# Autodesk Inventor assembly: Intake 1
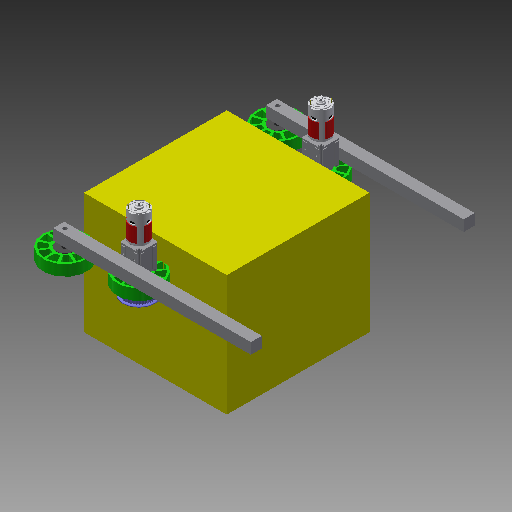
[picture p0: Inventor's stored thumbnail of the model, 512x512]
Saved by Autodesk Inventor 2018 (Build 220112000, 112)
## iProperties
Created: 2018-01-18
Part Number: Intake 1
Document SubType Name: Assembly
Designer: Apple
Author: Apple
## Documents named in this file (5)
- C:\Users\Apple\Documents\Inventor\2018 PowerUp\Cube Intake\Intake 1.iam
- C:\Users\Apple\Documents\Inventor\2018 PowerUp\2018 power cube.ipt
- C:\Users\Apple\Documents\Inventor\2018 PowerUp\Cube Intake\Sport57 with Redline and 4inc wheel.iam
- C:\Users\Apple\Documents\Inventor\2018 PowerUp\Cube Intake\Intake Arm.ipt
- C:\Users\Apple\Documents\Inventor\2018 PowerUp\AndyMark\am-3480+4IN+500Hex+Bore+Compliant+Wheel.ipt
## Components (7 placed, 4 different names)
1. 2018 power cube:1 — Mate:5, Mate:6, Flush:9
2. Sport57 with Redline and 4inc wheel:1 [sub-assembly] — Mate:1, Flush:2, Flush:3, Flush:4, Mate:6
3. Sport57 with Redline and 4inc wheel:2 [sub-assembly] — Mate:3, Flush:5, Flush:6, Mate:5, Mate:7
4. Intake Arm:1 — Mate:1, Flush:2, Flush:3, Mate:2, Flush:7, Flush:8
5. am-3480+4IN+500Hex+Bore+Compliant+Wheel:1 — Flush:4, Mate:2
6. Intake Arm:2 — Mate:3, Flush:5, Mate:4, Mate:7, Flush:7, Flush:8, Flush:9
7. am-3480+4IN+500Hex+Bore+Compliant+Wheel:2 — Mate:4, Flush:6
## Relationships (15: Flush 8, Mate 7)
- Mate:1: Sport57 with Redline and 4inc wheel:1 ↔ Intake Arm:1
- Flush:2: Sport57 with Redline and 4inc wheel:1 ↔ Intake Arm:1
- Flush:3 (127 mm): Sport57 with Redline and 4inc wheel:1 ↔ Intake Arm:1
- Flush:4: Sport57 with Redline and 4inc wheel:1 ↔ am-3480+4IN+500Hex+Bore+Compliant+Wheel:1
- Mate:2: Intake Arm:1 ↔ am-3480+4IN+500Hex+Bore+Compliant+Wheel:1
- Mate:3: Sport57 with Redline and 4inc wheel:2 ↔ Intake Arm:2
- Flush:5 (-127 mm): Sport57 with Redline and 4inc wheel:2 ↔ Intake Arm:2
- Mate:4: Intake Arm:2 ↔ am-3480+4IN+500Hex+Bore+Compliant+Wheel:2
- Flush:6: Sport57 with Redline and 4inc wheel:2 ↔ am-3480+4IN+500Hex+Bore+Compliant+Wheel:2
- Mate:5 (44.45 mm): 2018 power cube:1 ↔ Sport57 with Redline and 4inc wheel:2
- Mate:6 (44.45 mm): 2018 power cube:1 ↔ Sport57 with Redline and 4inc wheel:1
- Mate:7: Sport57 with Redline and 4inc wheel:2 ↔ Intake Arm:2
- Flush:7: Intake Arm:1 ↔ Intake Arm:2
- Flush:8: Intake Arm:1 ↔ Intake Arm:2
- Flush:9 (241.3 mm): 2018 power cube:1 ↔ Intake Arm:2
## Named parameters: CompliantCompress = 6.35 mm
